# Autodesk Inventor assembly: Pins
(part 2 of 2)
- C:\Users\cfang\Desktop\nebraska-silicon-lab\Hardware\ETL\modules\Tamale v1.6\etl_etroc_module_v44\VSS_D14_2.ipt
- C:\Users\cfang\Desktop\nebraska-silicon-lab\Hardware\ETL\modules\Tamale v1.6\etl_etroc_module_v44\VSS_D14_3.ipt
- C:\Users\cfang\Desktop\nebraska-silicon-lab\Hardware\ETL\modules\Tamale v1.6\etl_etroc_module_v44\VSS_D16.ipt
- C:\Users\cfang\Desktop\nebraska-silicon-lab\Hardware\ETL\modules\Tamale v1.6\etl_etroc_module_v44\VSS_D16_1.ipt
- C:\Users\cfang\Desktop\nebraska-silicon-lab\Hardware\ETL\modules\Tamale v1.6\etl_etroc_module_v44\VSS_D16_2.ipt
- C:\Users\cfang\Desktop\nebraska-silicon-lab\Hardware\ETL\modules\Tamale v1.6\etl_etroc_module_v44\VSS_D16_3.ipt
- C:\Users\cfang\Desktop\nebraska-silicon-lab\Hardware\ETL\modules\Tamale v1.6\etl_etroc_module_v44\VSS_D17.ipt
- C:\Users\cfang\Desktop\nebraska-silicon-lab\Hardware\ETL\modules\Tamale v1.6\etl_etroc_module_v44\VSS_D17_1.ipt
- C:\Users\cfang\Desktop\nebraska-silicon-lab\Hardware\ETL\modules\Tamale v1.6\etl_etroc_module_v44\VSS_D17_2.ipt
- C:\Users\cfang\Desktop\nebraska-silicon-lab\Hardware\ETL\modules\Tamale v1.6\etl_etroc_module_v44\VSS_D17_3.ipt
- C:\Users\cfang\Desktop\nebraska-silicon-lab\Hardware\ETL\modules\Tamale v1.6\etl_etroc_module_v44\VSS_D18.ipt
- C:\Users\cfang\Desktop\nebraska-silicon-lab\Hardware\ETL\modules\Tamale v1.6\etl_etroc_module_v44\VSS_D18_1.ipt
- C:\Users\cfang\Desktop\nebraska-silicon-lab\Hardware\ETL\modules\Tamale v1.6\etl_etroc_module_v44\VSS_D18_2.ipt
- C:\Users\cfang\Desktop\nebraska-silicon-lab\Hardware\ETL\modules\Tamale v1.6\etl_etroc_module_v44\VSS_D18_3.ipt
- C:\Users\cfang\Desktop\nebraska-silicon-lab\Hardware\ETL\modules\Tamale v1.6\etl_etroc_module_v44\VSS_D19.ipt
- C:\Users\cfang\Desktop\nebraska-silicon-lab\Hardware\ETL\modules\Tamale v1.6\etl_etroc_module_v44\VSS_D19_1.ipt
- C:\Users\cfang\Desktop\nebraska-silicon-lab\Hardware\ETL\modules\Tamale v1.6\etl_etroc_module_v44\VSS_D19_2.ipt
- C:\Users\cfang\Desktop\nebraska-silicon-lab\Hardware\ETL\modules\Tamale v1.6\etl_etroc_module_v44\VSS_D19_3.ipt
- C:\Users\cfang\Desktop\nebraska-silicon-lab\Hardware\ETL\modules\Tamale v1.6\etl_etroc_module_v44\VTEMP.ipt
- C:\Users\cfang\Desktop\nebraska-silicon-lab\Hardware\ETL\modules\Tamale v1.6\etl_etroc_module_v44\VTEMP_1.ipt
- C:\Users\cfang\Desktop\nebraska-silicon-lab\Hardware\ETL\modules\Tamale v1.6\etl_etroc_module_v44\VTEMP_2.ipt
- C:\Users\cfang\Desktop\nebraska-silicon-lab\Hardware\ETL\modules\Tamale v1.6\etl_etroc_module_v44\VTEMP_3.ipt
- C:\Users\cfang\Desktop\nebraska-silicon-lab\Hardware\ETL\modules\Tamale v1.6\etl_etroc_module_v44\WS_ADDR0.ipt
- C:\Users\cfang\Desktop\nebraska-silicon-lab\Hardware\ETL\modules\Tamale v1.6\etl_etroc_module_v44\WS_ADDR0_1.ipt
- C:\Users\cfang\Desktop\nebraska-silicon-lab\Hardware\ETL\modules\Tamale v1.6\etl_etroc_module_v44\WS_ADDR0_2.ipt
- C:\Users\cfang\Desktop\nebraska-silicon-lab\Hardware\ETL\modules\Tamale v1.6\etl_etroc_module_v44\WS_ADDR0_3.ipt
- C:\Users\cfang\Desktop\nebraska-silicon-lab\Hardware\ETL\modules\Tamale v1.6\etl_etroc_module_v44\WS_ADDR1.ipt
- C:\Users\cfang\Desktop\nebraska-silicon-lab\Hardware\ETL\modules\Tamale v1.6\etl_etroc_module_v44\WS_ADDR1_1.ipt
- C:\Users\cfang\Desktop\nebraska-silicon-lab\Hardware\ETL\modules\Tamale v1.6\etl_etroc_module_v44\WS_ADDR1_2.ipt
- C:\Users\cfang\Desktop\nebraska-silicon-lab\Hardware\ETL\modules\Tamale v1.6\etl_etroc_module_v44\WS_ADDR1_3.ipt
- C:\Users\cfang\Desktop\nebraska-silicon-lab\Hardware\ETL\modules\Tamale v1.6\etl_etroc_module_v44\WS_ADDR2.ipt
- C:\Users\cfang\Desktop\nebraska-silicon-lab\Hardware\ETL\modules\Tamale v1.6\etl_etroc_module_v44\WS_ADDR2_1.ipt
- C:\Users\cfang\Desktop\nebraska-silicon-lab\Hardware\ETL\modules\Tamale v1.6\etl_etroc_module_v44\WS_ADDR2_2.ipt
- C:\Users\cfang\Desktop\nebraska-silicon-lab\Hardware\ETL\modules\Tamale v1.6\etl_etroc_module_v44\WS_ADDR2_3.ipt
- C:\Users\cfang\Desktop\nebraska-silicon-lab\Hardware\ETL\modules\Tamale v1.6\etl_etroc_module_v44\WS_ADDR3.ipt
- C:\Users\cfang\Desktop\nebraska-silicon-lab\Hardware\ETL\modules\Tamale v1.6\etl_etroc_module_v44\WS_ADDR3_1.ipt
- C:\Users\cfang\Desktop\nebraska-silicon-lab\Hardware\ETL\modules\Tamale v1.6\etl_etroc_module_v44\WS_ADDR3_2.ipt
- C:\Users\cfang\Desktop\nebraska-silicon-lab\Hardware\ETL\modules\Tamale v1.6\etl_etroc_module_v44\WS_ADDR3_3.ipt
- C:\Users\cfang\Desktop\nebraska-silicon-lab\Hardware\ETL\modules\Tamale v1.6\etl_etroc_module_v44\WS_ADDR4.ipt
- C:\Users\cfang\Desktop\nebraska-silicon-lab\Hardware\ETL\modules\Tamale v1.6\etl_etroc_module_v44\WS_ADDR4_1.ipt
- C:\Users\cfang\Desktop\nebraska-silicon-lab\Hardware\ETL\modules\Tamale v1.6\etl_etroc_module_v44\WS_ADDR4_2.ipt
- C:\Users\cfang\Desktop\nebraska-silicon-lab\Hardware\ETL\modules\Tamale v1.6\etl_etroc_module_v44\WS_ADDR4_3.ipt
- C:\Users\cfang\Desktop\nebraska-silicon-lab\Hardware\ETL\modules\Tamale v1.6\etl_etroc_module_v44\WS_AVDD.ipt
- C:\Users\cfang\Desktop\nebraska-silicon-lab\Hardware\ETL\modules\Tamale v1.6\etl_etroc_module_v44\WS_AVDD_1.ipt
- C:\Users\cfang\Desktop\nebraska-silicon-lab\Hardware\ETL\modules\Tamale v1.6\etl_etroc_module_v44\WS_AVDD_2.ipt
- C:\Users\cfang\Desktop\nebraska-silicon-lab\Hardware\ETL\modules\Tamale v1.6\etl_etroc_module_v44\WS_AVDD_3.ipt
- C:\Users\cfang\Desktop\nebraska-silicon-lab\Hardware\ETL\modules\Tamale v1.6\etl_etroc_module_v44\WS_AVDD7.ipt
- C:\Users\cfang\Desktop\nebraska-silicon-lab\Hardware\ETL\modules\Tamale v1.6\etl_etroc_module_v44\WS_AVDD7_1.ipt
- C:\Users\cfang\Desktop\nebraska-silicon-lab\Hardware\ETL\modules\Tamale v1.6\etl_etroc_module_v44\WS_AVDD7_2.ipt
- C:\Users\cfang\Desktop\nebraska-silicon-lab\Hardware\ETL\modules\Tamale v1.6\etl_etroc_module_v44\WS_AVDD7_3.ipt
- C:\Users\cfang\Desktop\nebraska-silicon-lab\Hardware\ETL\modules\Tamale v1.6\etl_etroc_module_v44\WS_AVSS.ipt
- C:\Users\cfang\Desktop\nebraska-silicon-lab\Hardware\ETL\modules\Tamale v1.6\etl_etroc_module_v44\WS_AVSS_1.ipt
- C:\Users\cfang\Desktop\nebraska-silicon-lab\Hardware\ETL\modules\Tamale v1.6\etl_etroc_module_v44\WS_AVSS_2.ipt
- C:\Users\cfang\Desktop\nebraska-silicon-lab\Hardware\ETL\modules\Tamale v1.6\etl_etroc_module_v44\WS_AVSS_3.ipt
- C:\Users\cfang\Desktop\nebraska-silicon-lab\Hardware\ETL\modules\Tamale v1.6\etl_etroc_module_v44\WS_AVSS8.ipt
- C:\Users\cfang\Desktop\nebraska-silicon-lab\Hardware\ETL\modules\Tamale v1.6\etl_etroc_module_v44\WS_AVSS8_1.ipt
- C:\Users\cfang\Desktop\nebraska-silicon-lab\Hardware\ETL\modules\Tamale v1.6\etl_etroc_module_v44\WS_AVSS8_2.ipt
- C:\Users\cfang\Desktop\nebraska-silicon-lab\Hardware\ETL\modules\Tamale v1.6\etl_etroc_module_v44\WS_AVSS8_3.ipt
- C:\Users\cfang\Desktop\nebraska-silicon-lab\Hardware\ETL\modules\Tamale v1.6\etl_etroc_module_v44\WS_DVDD.ipt
- C:\Users\cfang\Desktop\nebraska-silicon-lab\Hardware\ETL\modules\Tamale v1.6\etl_etroc_module_v44\WS_DVDD_1.ipt
- C:\Users\cfang\Desktop\nebraska-silicon-lab\Hardware\ETL\modules\Tamale v1.6\etl_etroc_module_v44\WS_DVDD_2.ipt
- C:\Users\cfang\Desktop\nebraska-silicon-lab\Hardware\ETL\modules\Tamale v1.6\etl_etroc_module_v44\WS_DVDD_3.ipt
- C:\Users\cfang\Desktop\nebraska-silicon-lab\Hardware\ETL\modules\Tamale v1.6\etl_etroc_module_v44\WS_DVDD10.ipt
- C:\Users\cfang\Desktop\nebraska-silicon-lab\Hardware\ETL\modules\Tamale v1.6\etl_etroc_module_v44\WS_DVDD10_1.ipt
- C:\Users\cfang\Desktop\nebraska-silicon-lab\Hardware\ETL\modules\Tamale v1.6\etl_etroc_module_v44\WS_DVDD10_2.ipt
- C:\Users\cfang\Desktop\nebraska-silicon-lab\Hardware\ETL\modules\Tamale v1.6\etl_etroc_module_v44\WS_DVDD10_3.ipt
- C:\Users\cfang\Desktop\nebraska-silicon-lab\Hardware\ETL\modules\Tamale v1.6\etl_etroc_module_v44\WS_DVSS.ipt
- C:\Users\cfang\Desktop\nebraska-silicon-lab\Hardware\ETL\modules\Tamale v1.6\etl_etroc_module_v44\WS_DVSS_1.ipt
- C:\Users\cfang\Desktop\nebraska-silicon-lab\Hardware\ETL\modules\Tamale v1.6\etl_etroc_module_v44\WS_DVSS_2.ipt
- C:\Users\cfang\Desktop\nebraska-silicon-lab\Hardware\ETL\modules\Tamale v1.6\etl_etroc_module_v44\WS_DVSS_3.ipt
- C:\Users\cfang\Desktop\nebraska-silicon-lab\Hardware\ETL\modules\Tamale v1.6\etl_etroc_module_v44\WS_DVSS6.ipt
- C:\Users\cfang\Desktop\nebraska-silicon-lab\Hardware\ETL\modules\Tamale v1.6\etl_etroc_module_v44\WS_DVSS6_1.ipt
- C:\Users\cfang\Desktop\nebraska-silicon-lab\Hardware\ETL\modules\Tamale v1.6\etl_etroc_module_v44\WS_DVSS6_2.ipt
- C:\Users\cfang\Desktop\nebraska-silicon-lab\Hardware\ETL\modules\Tamale v1.6\etl_etroc_module_v44\WS_DVSS6_3.ipt
- C:\Users\cfang\Desktop\nebraska-silicon-lab\Hardware\ETL\modules\Tamale v1.6\etl_etroc_module_v44\WS_RSTN.ipt
- C:\Users\cfang\Desktop\nebraska-silicon-lab\Hardware\ETL\modules\Tamale v1.6\etl_etroc_module_v44\WS_RSTN_1.ipt
- C:\Users\cfang\Desktop\nebraska-silicon-lab\Hardware\ETL\modules\Tamale v1.6\etl_etroc_module_v44\WS_RSTN_2.ipt
- C:\Users\cfang\Desktop\nebraska-silicon-lab\Hardware\ETL\modules\Tamale v1.6\etl_etroc_module_v44\WS_RSTN_3.ipt
- C:\Users\cfang\Desktop\nebraska-silicon-lab\Hardware\ETL\modules\Tamale v1.6\etl_etroc_module_v44\WS_SCL.ipt
- C:\Users\cfang\Desktop\nebraska-silicon-lab\Hardware\ETL\modules\Tamale v1.6\etl_etroc_module_v44\WS_SCL_1.ipt
- C:\Users\cfang\Desktop\nebraska-silicon-lab\Hardware\ETL\modules\Tamale v1.6\etl_etroc_module_v44\WS_SCL_2.ipt
- C:\Users\cfang\Desktop\nebraska-silicon-lab\Hardware\ETL\modules\Tamale v1.6\etl_etroc_module_v44\WS_SCL_3.ipt
- C:\Users\cfang\Desktop\nebraska-silicon-lab\Hardware\ETL\modules\Tamale v1.6\etl_etroc_module_v44\WS_SDA.ipt
- C:\Users\cfang\Desktop\nebraska-silicon-lab\Hardware\ETL\modules\Tamale v1.6\etl_etroc_module_v44\WS_SDA_1.ipt
- C:\Users\cfang\Desktop\nebraska-silicon-lab\Hardware\ETL\modules\Tamale v1.6\etl_etroc_module_v44\WS_SDA_2.ipt
- C:\Users\cfang\Desktop\nebraska-silicon-lab\Hardware\ETL\modules\Tamale v1.6\etl_etroc_module_v44\WS_SDA_3.ipt
- C:\Users\cfang\Desktop\nebraska-silicon-lab\Hardware\ETL\modules\Tamale v1.6\etl_etroc_module_v44\WS_WR_EN.ipt
- C:\Users\cfang\Desktop\nebraska-silicon-lab\Hardware\ETL\modules\Tamale v1.6\etl_etroc_module_v44\WS_WR_EN_1.ipt
- C:\Users\cfang\Desktop\nebraska-silicon-lab\Hardware\ETL\modules\Tamale v1.6\etl_etroc_module_v44\WS_WR_EN_2.ipt
- C:\Users\cfang\Desktop\nebraska-silicon-lab\Hardware\ETL\modules\Tamale v1.6\etl_etroc_module_v44\WS_WR_EN_3.ipt
## Components (538 placed, 143 different names)
1. 1
2. 1:1
3. 1:2
4. 1:3
5. 1:4
6. 1:5
7. 1:6
8. 1:7
9. 1:8
10. 1:9
11. 1:10
12. 1:11
13. 1:12
14. 1:13
15. 1:14
16. 1:15
17. 1:16
18. 1:17
19. 1:18
20. 1:19
21. 1:20
22. 1:21
23. 1:22
24. 1:23
25. 1:24
26. 1:25
27. 1:26
28. 1:27
29. 1:28
30. 1:29
31. 1:30
32. 1:31
33. 1:32
34. 1:33
35. 1:34
36. 1:35
37. 1:36
38. 1:37
39. 1:38
40. 1:39
41. 1:40
42. 1:41
43. 1:42
44. 1:43
45. 1:44
46. 1:45
47. 1:46
48. 1:47
49. 1:48
50. 1:49
51. 1:50
52. 1:51
53. 1:52
54. 1:53
55. 1:54
56. 1:55
57. 1:56
58. 1:57
59. 1:58
60. 1:59
61. 1:60
62. 1:61
63. 1:62
64. 1:63
65. 1:64
66. 1:65
67. 1:66
68. 1:67
69. 1:68
70. 1:69
71. 1:70
72. 1:71
73. 1:72
74. 1:73
75. 1:74
76. 1:75
77. 1:76
78. 1:77
79. 1:78
80. 1:79
81. 1:80
82. 1:81
83. 1:82
84. 1:83
85. 1:84
86. 1:85
87. 1:86
88. 1:87
89. 1:88
90. 1:89
91. 1:90
92. 1:91
93. 1:92
94. 1:93
95. 1:94
96. 1:95
97. 1:96
98. 1:97
99. 1:98
100. 1:99
101. 1:100
102. 1:101
103. 1:102
104. 10
105. 11
106. 12
107. 13
108. 14
109. 15
110. 16
111. 17
112. 18
113. 19
114. 2
115. 2:1
116. 2:2
117. 2:3
118. 2:4
119. 2:5
120. 2:6
121. 2:7
122. 2:8
123. 2:9
124. 2:10
125. 2:11
126. 2:12
127. 2:13
128. 2:14
129. 2:15
130. 2:16
131. 2:17
132. 2:18
133. 2:19
134. 2:20
135. 2:21
136. 2:22
137. 2:23
138. 2:24
139. 2:25
140. 2:26
141. 2:27
142. 2:28
143. 2:29
144. 2:30
145. 2:31
146. 2:32
147. 2:33
148. 2:34
149. 2:35
150. 2:36
151. 2:37
152. 2:38
153. 2:39
154. 2:40
155. 2:41
156. 2:42
157. 2:43
158. 2:44
159. 2:45
160. 2:46
161. 2:47
162. 2:48
163. 2:49
164. 2:50
165. 2:51
166. 2:52
167. 2:53
168. 2:54
169. 2:55
170. 2:56
171. 2:57
172. 2:58
173. 2:59
174. 2:60
175. 2:61
176. 2:62
177. 2:63
178. 2:64
179. 2:65
180. 2:66
181. 2:67
182. 2:68
183. 2:69
184. 2:70
185. 2:71
186. 2:72
187. 2:73
188. 2:74
189. 2:75
190. 2:76
191. 2:77
192. 2:78
193. 2:79
194. 2:80
195. 2:81
196. 2:82
197. 2:83
198. 2:84
199. 2:85
200. 2:86
201. 2:87
202. 2:88
203. 2:89
204. 2:90
205. 2:91
206. 2:92
207. 2:93
208. 2:94
209. 2:95
210. 2:96
211. 2:97
212. 2:98
213. 2:99
214. 2:100
215. 2:101
216. 2:102
217. 20
218. 21
219. 22
220. 23
221. 24
222. 25
223. 26
224. 27
225. 28
226. 29
227. 3
228. 3:1
229. 3:2
230. 30
231. 31
232. 32
233. 33
234. 34
235. 35
236. 36
237. 37
238. 38
239. 39
240. 4
241. 40
242. 41
243. 42
244. 43
245. 44
246. 45
247. 46
248. 47
249. 48
250. 49
251. 5
252. 50
253. 51
254. 52
255. 53
256. 54
257. 55
258. 56
259. 57
260. 58
261. 59
262. 6
263. 60
264. 61
265. 62
266. 63
267. 64
268. 65
269. 66
270. 67
271. 68
272. 69
273. 7
274. 70
275. 71
276. 72
277. 73
278. 74
279. 75
280. 76
281. 77
282. 78
283. 8
284. 9
285. CLK1280_N
286. CLK1280_N:1
287. CLK1280_N:2
288. CLK1280_N:3
289. CLK1280_P
290. CLK1280_P:1
291. CLK1280_P:2
292. CLK1280_P:3
293. CLK40_N
294. CLK40_N:1
295. CLK40_N:2
296. CLK40_N:3
297. CLK40_P
298. CLK40_P:1
299. CLK40_P:2
300. CLK40_P:3
301. DOL_N
302. DOL_N:1
303. DOL_N:2
304. DOL_N:3
305. DOL_P
306. DOL_P:1
307. DOL_P:2
308. DOL_P:3
309. DOR_N
310. DOR_N:1
311. DOR_N:2
312. DOR_N:3
313. DOR_P
314. DOR_P:1
315. DOR_P:2
316. DOR_P:3
317. FCN
318. FCN:1
319. FCN:2
320. FCN:3
321. FCP
322. FCP:1
323. FCP:2
324. FCP:3
325. I2C_ADDR0
326. I2C_ADDR0:1
327. I2C_ADDR0:2
328. I2C_ADDR0:3
329. I2C_ADDR1
330. I2C_ADDR1:1
331. I2C_ADDR1:2
332. I2C_ADDR1:3
333. I2C_ADDR2
334. I2C_ADDR2:1
335. I2C_ADDR2:2
336. I2C_ADDR2:3
337. I2C_ADDR3
338. I2C_ADDR3:1
339. I2C_ADDR3:2
340. I2C_ADDR3:3
341. I2C_ADDR4
342. I2C_ADDR4:1
343. I2C_ADDR4:2
344. I2C_ADDR4:3
345. POWER1
346. POWER2
347. RSTN
348. RSTN:1
349. RSTN:2
350. RSTN:3
351. SCL
352. SCL:1
353. SCL:2
354. SCL:3
355. SDA
356. SDA:1
357. SDA:2
358. SDA:3
359. TP
360. TP:1
361. TP:2
362. TP:3
363. VDD_A
364. VDD_A:1
365. VDD_A:2
366. VDD_A:3
367. VDD_A1
368. VDD_A1:1
369. VDD_A1:2
370. VDD_A1:3
371. VDD_A12
372. VDD_A12:1
373. VDD_A12:2
374. VDD_A12:3
375. VDD_A5
376. VDD_A5:1
377. VDD_A5:2
378. VDD_A5:3
379. VDD_D
380. VDD_D:1
381. VDD_D:2
382. VDD_D:3
383. VDD_D11
384. VDD_D11:1
385. VDD_D11:2
386. VDD_D11:3
387. VDD_D15
388. VDD_D15:1
389. VDD_D15:2
390. VDD_D15:3
391. VDD_D20
392. VDD_D20:1
393. VDD_D20:2
394. VDD_D20:3
395. VDD_D21
396. VDD_D21:1
397. VDD_D21:2
398. VDD_D21:3
399. VDD_EFUSE
400. VDD_EFUSE:1
401. VDD_EFUSE:2
402. VDD_EFUSE:3
403. VP
404. VP:1
405. VP:2
406. VP:3
407. VREF
408. VREF:1
409. VREF:2
410. VREF:3
411. VSS_A
412. VSS_A:1
413. VSS_A:2
414. VSS_A:3
415. VSS_A2
416. VSS_A2:1
417. VSS_A2:2
418. VSS_A2:3
419. VSS_A22
420. VSS_A22:1
421. VSS_A22:2
422. VSS_A22:3
423. VSS_A3
424. VSS_A3:1
425. VSS_A3:2
426. VSS_A3:3
427. VSS_A4
428. VSS_A4:1
429. VSS_A4:2
430. VSS_A4:3
431. VSS_A9
432. VSS_A9:1
433. VSS_A9:2
434. VSS_A9:3
435. VSS_AO
436. VSS_AO:1
437. VSS_AO:2
438. VSS_AO:3
439. VSS_D
440. VSS_D:1
441. VSS_D:2
442. VSS_D:3
443. VSS_D13
444. VSS_D13:1
445. VSS_D13:2
446. VSS_D13:3
447. VSS_D14
448. VSS_D14:1
449. VSS_D14:2
450. VSS_D14:3
451. VSS_D16
452. VSS_D16:1
453. VSS_D16:2
454. VSS_D16:3
455. VSS_D17
456. VSS_D17:1
457. VSS_D17:2
458. VSS_D17:3
459. VSS_D18
460. VSS_D18:1
461. VSS_D18:2
462. VSS_D18:3
463. VSS_D19
464. VSS_D19:1
465. VSS_D19:2
466. VSS_D19:3
467. VTEMP
468. VTEMP:1
469. VTEMP:2
470. VTEMP:3
471. WS_ADDR0
472. WS_ADDR0:1
473. WS_ADDR0:2
474. WS_ADDR0:3
475. WS_ADDR1
476. WS_ADDR1:1
477. WS_ADDR1:2
478. WS_ADDR1:3
479. WS_ADDR2
480. WS_ADDR2:1
481. WS_ADDR2:2
482. WS_ADDR2:3
483. WS_ADDR3
484. WS_ADDR3:1
485. WS_ADDR3:2
486. WS_ADDR3:3
487. WS_ADDR4
488. WS_ADDR4:1
489. WS_ADDR4:2
490. WS_ADDR4:3
491. WS_AVDD
492. WS_AVDD:1
493. WS_AVDD:2
494. WS_AVDD:3
495. WS_AVDD7
496. WS_AVDD7:1
497. WS_AVDD7:2
498. WS_AVDD7:3
499. WS_AVSS
500. WS_AVSS:1
501. WS_AVSS:2
502. WS_AVSS:3
503. WS_AVSS8
504. WS_AVSS8:1
505. WS_AVSS8:2
506. WS_AVSS8:3
507. WS_DVDD
508. WS_DVDD:1
509. WS_DVDD:2
510. WS_DVDD:3
511. WS_DVDD10
512. WS_DVDD10:1
513. WS_DVDD10:2
514. WS_DVDD10:3
515. WS_DVSS
516. WS_DVSS:1
517. WS_DVSS:2
518. WS_DVSS:3
519. WS_DVSS6
520. WS_DVSS6:1
521. WS_DVSS6:2
522. WS_DVSS6:3
523. WS_RSTN
524. WS_RSTN:1
525. WS_RSTN:2
526. WS_RSTN:3
527. WS_SCL
528. WS_SCL:1
529. WS_SCL:2
530. WS_SCL:3
531. WS_SDA
532. WS_SDA:1
533. WS_SDA:2
534. WS_SDA:3
535. WS_WR_EN
536. WS_WR_EN:1
537. WS_WR_EN:2
538. WS_WR_EN:3
